# Autodesk Inventor assembly: WindowMotorMounting
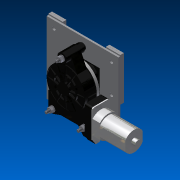
[picture p0: Inventor's stored thumbnail of the model, 180x180]
Saved by Autodesk Inventor 2013 (Build 170138000, 138)
## iProperties
Created: 2013-07-16
Part Number: WindowMotorMounting
Document SubType Name: Assembly
Designer: orange
Author: orange
## Documents named in this file (10)
- I:\FRC_Projects\Cad\Inventor_Projects\Shooter_No_Welding\Hopper\WindowMotorMounting.iam
- I:\FRC_Projects\Cad\Inventor_Projects\Shooter_No_Welding\UnmoddedKOP\MOT_WindowMotor_262100-3040.ipt
- I:\FRC_Projects\Cad\Inventor_Projects\Shooter_No_Welding\Hopper\Window_MotorMounting.ipt
- I:\FRC_Projects\Cad\Inventor_Projects\Shooter_No_Welding\Hopper\MOT_Coupler_Denso-6.ipt
- I:\FRC_Projects\Cad\Inventor_Projects\Shooter_No_Welding\Library\AS 1110 - M5 x 50.ipt
- I:\FRC_Projects\Cad\Inventor_Projects\Shooter_No_Welding\Library\AS 1110 - M5 x 40.ipt
- I:\FRC_Projects\Cad\Inventor_Projects\Shooter_No_Welding\Library\AS 1112 - M5  Type 5.ipt
- I:\FRC_Projects\Cad\Inventor_Projects\Shooter_No_Welding\Library\AS 1971 - 5(1).ipt
- I:\FRC_Projects\Cad\Inventor_Projects\Shooter_No_Welding\Hopper\Spacer.ipt
- I:\FRC_Projects\Cad\Inventor_Projects\Shooter_No_Welding\Hopper\Spacer$in.ipt
## Components (16 placed, 9 different names)
1. MOT_WindowMotor_262100-3040:1 — Mate:4, Mate:5, Mate:6, Mate:7, Mate:8, Mate:9, Mate:22, Mate:25, Mate:28
2. Window_MotorMounting:1 — Mate:4, Mate:5, Mate:6, Mate:7, Mate:10, Mate:11, Mate:16, Mate:17, Mate:18, Mate:19, Mate:43, Mate:49
3. MOT_Coupler_Denso-6:1 — Mate:8, Mate:9
4. AS 1110 - Metric M5 x 50:1 — Mate:10, Mate:11, Mate:20, Mate:21, Mate:23
5. AS 1110 - Metric M5 x 40:1 — Mate:16, Mate:17, Mate:26, Mate:32
6. AS 1110 - Metric M5 x 40:2 — Mate:18, Mate:19, Mate:27, Mate:29
7. AS 1112 (2) - Metric M5  Type 5:1 — Mate:20, Mate:23, Mate:24
8. AS 1112 (2) - Metric M5  Type 5:2 — Mate:31, Mate:32
9. AS 1112 (2) - Metric M5  Type 5:3 — Mate:29, Mate:30
10. AS 1971 (M - 5) 5:1 — Mate:21, Mate:22, Mate:24
11. AS 1971 (M - 5) 5:2 — Mate:25, Mate:26, Mate:31
12. AS 1971 (M - 5) 5:3 — Mate:27, Mate:28, Mate:30
13. Spacer:1 — Mate:43, Mate:44
14. Spacer:2 — Mate:44
15. Spacer$in:1 — Mate:49, Mate:52
16. Spacer$in:2 — Mate:52
## Relationships (29: Mate 29)
- Mate:4: MOT_WindowMotor_262100-3040:1 ↔ Window_MotorMounting:1
- Mate:5: MOT_WindowMotor_262100-3040:1 ↔ Window_MotorMounting:1
- Mate:6: MOT_WindowMotor_262100-3040:1 ↔ Window_MotorMounting:1
- Mate:7: MOT_WindowMotor_262100-3040:1 ↔ Window_MotorMounting:1
- Mate:8: MOT_WindowMotor_262100-3040:1 ↔ MOT_Coupler_Denso-6:1
- Mate:9: MOT_WindowMotor_262100-3040:1 ↔ MOT_Coupler_Denso-6:1
- Mate:10: Window_MotorMounting:1 ↔ AS 1110 - Metric M5 x 50:1
- Mate:11: Window_MotorMounting:1 ↔ AS 1110 - Metric M5 x 50:1
- Mate:16: Window_MotorMounting:1 ↔ AS 1110 - Metric M5 x 40:1
- Mate:17: Window_MotorMounting:1 ↔ AS 1110 - Metric M5 x 40:1
- Mate:18: Window_MotorMounting:1 ↔ AS 1110 - Metric M5 x 40:2
- Mate:19: Window_MotorMounting:1 ↔ AS 1110 - Metric M5 x 40:2
- Mate:20: AS 1110 - Metric M5 x 50:1 ↔ AS 1112 (2) - Metric M5  Type 5:1
- Mate:21: AS 1110 - Metric M5 x 50:1 ↔ AS 1971 (M - 5) 5:1
- Mate:22: MOT_WindowMotor_262100-3040:1 ↔ AS 1971 (M - 5) 5:1
- Mate:23: AS 1110 - Metric M5 x 50:1 ↔ AS 1112 (2) - Metric M5  Type 5:1
- Mate:24: AS 1112 (2) - Metric M5  Type 5:1 ↔ AS 1971 (M - 5) 5:1
- Mate:25: MOT_WindowMotor_262100-3040:1 ↔ AS 1971 (M - 5) 5:2
- Mate:26: AS 1110 - Metric M5 x 40:1 ↔ AS 1971 (M - 5) 5:2
- Mate:27: AS 1110 - Metric M5 x 40:2 ↔ AS 1971 (M - 5) 5:3
- Mate:28: MOT_WindowMotor_262100-3040:1 ↔ AS 1971 (M - 5) 5:3
- Mate:29: AS 1110 - Metric M5 x 40:2 ↔ AS 1112 (2) - Metric M5  Type 5:3
- Mate:30: AS 1112 (2) - Metric M5  Type 5:3 ↔ AS 1971 (M - 5) 5:3
- Mate:31: AS 1112 (2) - Metric M5  Type 5:2 ↔ AS 1971 (M - 5) 5:2
- Mate:32: AS 1110 - Metric M5 x 40:1 ↔ AS 1112 (2) - Metric M5  Type 5:2
- Mate:43: Window_MotorMounting:1 ↔ Spacer:1
- Mate:44: Spacer:1 ↔ Spacer:2
- Mate:49: Window_MotorMounting:1 ↔ Spacer$in:1
- Mate:52: Spacer$in:1 ↔ Spacer$in:2
